# Autodesk Inventor assembly: 조립
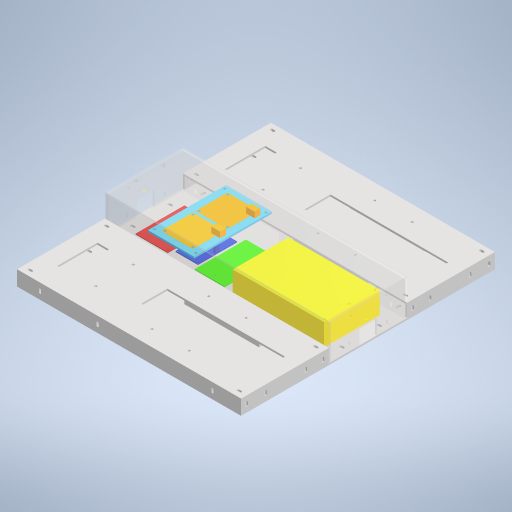
[picture p0: Inventor's stored thumbnail of the model, 512x512]
Saved by Autodesk Inventor 2024 (Build 280153000, 153)
## iProperties
Created: 2024-04-10
Part Number: 조립
Document SubType Name: Assembly
Designer: ckhye
Author: ckhye
## iProperties of the stored document 라즈베리파이.ipt
Created: 2024-06-01
Part Number: 라즈베리파이
Material: Generic
Document SubType Name: Modeling
Designer: ckhye
Density: 1 g/cm^3
Appearance: 기본값
Sending System: Autodesk Inventor 2025
Author: ckhye
## iProperties of the stored document 모터드라이버.ipt
Created: 2024-06-01
Part Number: 모터드라이버
Material: Generic
Document SubType Name: Modeling
Designer: ckhye
Density: 1 g/cm^3
Appearance: 기본값
Sending System: Autodesk Inventor 2025
Author: ckhye
## iProperties of the stored document 컨버터.ipt
Created: 2024-06-01
Part Number: 컨버터
Material: Generic
Document SubType Name: Modeling
Designer: ckhye
Density: 1 g/cm^3
Appearance: 기본값
Sending System: Autodesk Inventor 2025
Author: ckhye
## iProperties of the stored document SMPS.ipt
Created: 2024-06-01
Part Number: SMPS
Material: Generic
Document SubType Name: Modeling
Designer: ckhye
Density: 1 g/cm^3
Appearance: 기본값
Sending System: Autodesk Inventor 2025
Author: ckhye
## iProperties of the stored document 빵판.ipt
Created: 2024-06-01
Part Number: 빵판
Material: Generic
Document SubType Name: Modeling
Designer: ckhye
Density: 1 g/cm^3
Appearance: 기본값
Sending System: Autodesk Inventor 2025
Author: ckhye
## Documents named in this file (20)
- C:\Users\kkamin5\OneDrive - UOS\문서\Inventor\EBS project\모델링최종\조립.iam
- C:\Users\kkamin5\OneDrive - UOS\문서\Inventor\EBS project\모델링최종\발 받침대 받침_밑면.ipt
- C:\Users\kkamin5\OneDrive - UOS\문서\Inventor\EBS project\모델링최종\발 받침대 받침_위,아래.ipt
- C:\Users\kkamin5\OneDrive - UOS\문서\Inventor\EBS project\모델링최종\발 받침대 받침_좌,우.ipt
- C:\Users\kkamin5\OneDrive - UOS\문서\Inventor\EBS project\모델링최종\3D지지대.ipt
- C:\Users\kkamin5\OneDrive - UOS\문서\Inventor\EBS project\모델링최종\라즈베리파이보관_옆판.ipt
- C:\Users\kkamin5\OneDrive - UOS\문서\Inventor\EBS project\모델링최종\발받침대받침옆판.ipt
- C:\Users\kkamin5\OneDrive - UOS\문서\Inventor\EBS project\모델링최종\라즈베리파이보관_윗판.ipt
- C:\Users\kkamin5\OneDrive - UOS\문서\Inventor\EBS project\모델링최종\발 받침대 받침_윗면.ipt
- **C:\Users\kkamin5\OneDrive - UOS\문서\Inventor\EBS project\모델링최종\조립.iam*LocalDocs*xAaaaatbaAaaaaaaaAaaaqs4bRc*SMPS.ipt
- **C:\Users\kkamin5\OneDrive - UOS\문서\Inventor\EBS project\모델링최종\조립.iam*LocalDocs*xAaaaakbaAaaaaaaaAaaaqwuvSe*라즈베리파이.ipt
- **C:\Users\kkamin5\OneDrive - UOS\문서\Inventor\EBS project\모델링최종\조립.iam*LocalDocs*xAaaaqkbaAaaaaaaaAaaaamyz2g*빵판.ipt
- **C:\Users\kkamin5\OneDrive - UOS\문서\Inventor\EBS project\모델링최종\조립.iam*LocalDocs*xAaaaajbaAaaaaaaaAaaaag3xYb*모터드라이버.ipt
- **C:\Users\kkamin5\OneDrive - UOS\문서\Inventor\EBS project\모델링최종\조립.iam*LocalDocs*xAaaaqjbaAaaaaaaaAaaaqjrfGf*컨버터.ipt
- C:\Users\kkamin5\OneDrive - UOS\문서\Inventor\EBS project\모델링최종\라즈베리파이 보관소 2층 판.ipt
- C:\Users\kkamin5\OneDrive - UOS\문서\Inventor\EBS project\모델링최종\SMPS.ipt
- C:\Users\kkamin5\OneDrive - UOS\문서\Inventor\EBS project\모델링최종\라즈베리파이.ipt
- C:\Users\kkamin5\OneDrive - UOS\문서\Inventor\EBS project\모델링최종\빵판.ipt
- C:\Users\kkamin5\OneDrive - UOS\문서\Inventor\EBS project\모델링최종\모터드라이버.ipt
- C:\Users\kkamin5\OneDrive - UOS\문서\Inventor\EBS project\모델링최종\컨버터.ipt
## Components (27 placed, 14 different names)
1. 발 받침대 받침_밑면:1 — 메이트:1, 플러쉬:1, 메이트:2, 메이트:3, 플러쉬:3, 메이트:4, 플러쉬:5, 메이트:5, 플러쉬:6, 플러쉬:8, 메이트:7, 메이트:8, 플러쉬:10, 플러쉬:11, 플러쉬:12, 플러쉬:13, 메이트:13, 메이트:14, 메이트:15, 메이트:16, 메이트:17, 메이트:18, 메이트:35, 메이트:36, 메이트:38, 플러쉬:20, 플러쉬:22, 플러쉬:23, 메이트:67, 메이트:69, 메이트:76, 메이트:87, 메이트:92, 메이트:93, 메이트:94, 메이트:95, 메이트:96, 메이트:97, 메이트:98, 메이트:99, 메이트:100, 메이트:101, 메이트:102, 메이트:103
2. 발 받침대 받침_위,아래:1 — 메이트:3, 플러쉬:3, 메이트:10, 메이트:19
3. 발 받침대 받침_위,아래:2 — 메이트:4, 플러쉬:5, 메이트:9, 메이트:50
4. 발 받침대 받침_위,아래:3 — 메이트:5, 플러쉬:6, 메이트:12, 메이트:54, 플러쉬:30
5. 발 받침대 받침_위,아래:4 — 플러쉬:8, 메이트:27, 메이트:87, 메이트:88
6. 발 받침대 받침_좌,우:2 — 메이트:8, 플러쉬:12, 플러쉬:13, 메이트:12, 메이트:29, 플러쉬:29, 메이트:88
7. 발 받침대 받침_좌,우:4 — 메이트:7, 플러쉬:10, 플러쉬:11, 메이트:9, 메이트:10, 메이트:24, 메이트:53, 플러쉬:26, 플러쉬:27
8. 3D지지대:1 — 메이트:14, 메이트:60, 메이트:61
9. 3D지지대:2 — 메이트:16, 메이트:27, 메이트:29
10. 3D지지대:3 — 메이트:13, 메이트:62, 메이트:63
11. 3D지지대:4 — 메이트:17, 메이트:56, 메이트:57
12. 3D지지대:5 — 메이트:15, 메이트:58, 메이트:59
13. 3D지지대:6 — 메이트:18, 메이트:19, 메이트:24
14. 라즈베리파이보관_옆판:1 — 메이트:35, 플러쉬:22, 메이트:50, 플러쉬:25, 메이트:55, 메이트:84, 플러쉬:34, 플러쉬:35, 메이트:91
15. 라즈베리파이보관_옆판:2 — 메이트:36, 플러쉬:23, 메이트:52, 메이트:78, 메이트:83, 플러쉬:38
16. 발받침대받침옆판:1 — 메이트:38, 플러쉬:20, 메이트:55, 플러쉬:33
17. 라즈베리파이보관_윗판:1 — 메이트:52, 플러쉬:25, 메이트:85, 플러쉬:36
18. 발 받침대 받침_윗면:1 — 메이트:54, 플러쉬:29, 플러쉬:30, 메이트:60, 메이트:61, 메이트:62, 메이트:63
19. 발받침대받침옆판:2 — 메이트:83, 메이트:84, 플러쉬:34, 플러쉬:35, 메이트:85, 메이트:86, 플러쉬:36
20. SMPS:1 — 메이트:67, 메이트:78, 메이트:86
21. 라즈베리파이:1 — 메이트:69, 메이트:92, 메이트:93, 메이트:94, 메이트:95
22. 빵판:1 — 메이트:101, 메이트:102, 메이트:103
23. 모터드라이버:1 — 메이트:77, 플러쉬:32, 메이트:90
24. 컨버터:1 — 메이트:96, 메이트:97, 메이트:98, 메이트:99, 메이트:100
25. 라즈베리파이 보관소 2층 판:1 — 메이트:76, 메이트:77, 플러쉬:32, 플러쉬:33, 메이트:89, 플러쉬:37, 플러쉬:38
26. 모터드라이버:2 — 메이트:89, 플러쉬:37, 메이트:90, 메이트:91
27. 발 받침대 받침_윗면:2 — 메이트:53, 플러쉬:26, 플러쉬:27, 메이트:56, 메이트:57, 메이트:58, 메이트:59
## Relationships (86: Mate 62, Flush 24)
- 메이트:1 [Mate]: 발 받침대 받침_밑면:1
- 플러쉬:1 [Flush]: 발 받침대 받침_밑면:1
- 메이트:2 [Mate]: 발 받침대 받침_밑면:1
- 메이트:3 [Mate]: 발 받침대 받침_밑면:1 ↔ 발 받침대 받침_위,아래:1
- 플러쉬:3 [Flush]: 발 받침대 받침_밑면:1 ↔ 발 받침대 받침_위,아래:1
- 메이트:4 [Mate]: 발 받침대 받침_밑면:1 ↔ 발 받침대 받침_위,아래:2
- 플러쉬:5 [Flush]: 발 받침대 받침_밑면:1 ↔ 발 받침대 받침_위,아래:2
- 메이트:5 [Mate]: 발 받침대 받침_밑면:1 ↔ 발 받침대 받침_위,아래:3
- 플러쉬:6 [Flush]: 발 받침대 받침_밑면:1 ↔ 발 받침대 받침_위,아래:3
- 플러쉬:8 [Flush]: 발 받침대 받침_밑면:1 ↔ 발 받침대 받침_위,아래:4
- 메이트:7 [Mate]: 발 받침대 받침_밑면:1 ↔ 발 받침대 받침_좌,우:4
- 메이트:8 [Mate]: 발 받침대 받침_밑면:1 ↔ 발 받침대 받침_좌,우:2
- 플러쉬:10 [Flush]: 발 받침대 받침_밑면:1 ↔ 발 받침대 받침_좌,우:4
- 플러쉬:11 [Flush]: 발 받침대 받침_밑면:1 ↔ 발 받침대 받침_좌,우:4
- 플러쉬:12 [Flush]: 발 받침대 받침_밑면:1 ↔ 발 받침대 받침_좌,우:2
- 플러쉬:13 [Flush]: 발 받침대 받침_밑면:1 ↔ 발 받침대 받침_좌,우:2
- 메이트:9 [Mate]: 발 받침대 받침_위,아래:2 ↔ 발 받침대 받침_좌,우:4
- 메이트:10 [Mate]: 발 받침대 받침_위,아래:1 ↔ 발 받침대 받침_좌,우:4
- 메이트:12 [Mate]: 발 받침대 받침_위,아래:3 ↔ 발 받침대 받침_좌,우:2
- 메이트:13 [Mate]: 발 받침대 받침_밑면:1 ↔ 3D지지대:3
- 메이트:14 [Mate]: 발 받침대 받침_밑면:1 ↔ 3D지지대:1
- 메이트:15 [Mate]: 발 받침대 받침_밑면:1 ↔ 3D지지대:5
- 메이트:16 [Mate]: 발 받침대 받침_밑면:1 ↔ 3D지지대:2
- 메이트:17 [Mate]: 발 받침대 받침_밑면:1 ↔ 3D지지대:4
- 메이트:18 [Mate]: 발 받침대 받침_밑면:1 ↔ 3D지지대:6
- 메이트:19 [Mate] (81 mm): 발 받침대 받침_위,아래:1 ↔ 3D지지대:6
- 메이트:24 [Mate] (7.5 mm): 발 받침대 받침_좌,우:4 ↔ 3D지지대:6
- 메이트:27 [Mate] (81 mm): 발 받침대 받침_위,아래:4 ↔ 3D지지대:2
- 메이트:29 [Mate] (7.5 mm): 발 받침대 받침_좌,우:2 ↔ 3D지지대:2
- 메이트:35 [Mate]: 발 받침대 받침_밑면:1 ↔ 라즈베리파이보관_옆판:1
- 메이트:36 [Mate]: 발 받침대 받침_밑면:1 ↔ 라즈베리파이보관_옆판:2
- 메이트:38 [Mate]: 발 받침대 받침_밑면:1 ↔ 발받침대받침옆판:1
- 플러쉬:20 [Flush]: 발 받침대 받침_밑면:1 ↔ 발받침대받침옆판:1
- 플러쉬:22 [Flush]: 발 받침대 받침_밑면:1 ↔ 라즈베리파이보관_옆판:1
- 메이트:50 [Mate]: 발 받침대 받침_위,아래:2 ↔ 라즈베리파이보관_옆판:1
- 플러쉬:23 [Flush]: 발 받침대 받침_밑면:1 ↔ 라즈베리파이보관_옆판:2
- 메이트:52 [Mate]: 라즈베리파이보관_옆판:2 ↔ 라즈베리파이보관_윗판:1
- 플러쉬:25 [Flush]: 라즈베리파이보관_옆판:1 ↔ 라즈베리파이보관_윗판:1
- 메이트:53 [Mate]: 발 받침대 받침_좌,우:4 ↔ 발 받침대 받침_윗면:2
- 플러쉬:26 [Flush]: 발 받침대 받침_좌,우:4 ↔ 발 받침대 받침_윗면:2
- 플러쉬:27 [Flush]: 발 받침대 받침_좌,우:4 ↔ 발 받침대 받침_윗면:2
- 메이트:54 [Mate]: 발 받침대 받침_위,아래:3 ↔ 발 받침대 받침_윗면:1
- 플러쉬:29 [Flush]: 발 받침대 받침_좌,우:2 ↔ 발 받침대 받침_윗면:1
- 플러쉬:30 [Flush]: 발 받침대 받침_위,아래:3 ↔ 발 받침대 받침_윗면:1
- 메이트:55 [Mate]: 라즈베리파이보관_옆판:1 ↔ 발받침대받침옆판:1
- 메이트:56 [Mate]: 3D지지대:4 ↔ 발 받침대 받침_윗면:2
- 메이트:57 [Mate]: 3D지지대:4 ↔ 발 받침대 받침_윗면:2
- 메이트:58 [Mate]: 3D지지대:5 ↔ 발 받침대 받침_윗면:2
- 메이트:59 [Mate]: 3D지지대:5 ↔ 발 받침대 받침_윗면:2
- 메이트:60 [Mate]: 3D지지대:1 ↔ 발 받침대 받침_윗면:1
- 메이트:61 [Mate]: 3D지지대:1 ↔ 발 받침대 받침_윗면:1
- 메이트:62 [Mate]: 3D지지대:3 ↔ 발 받침대 받침_윗면:1
- 메이트:63 [Mate]: 3D지지대:3 ↔ 발 받침대 받침_윗면:1
- 메이트:67 [Mate]: 발 받침대 받침_밑면:1 ↔ SMPS:1
- 메이트:69 [Mate]: 발 받침대 받침_밑면:1 ↔ 라즈베리파이:1
- 메이트:76 [Mate] (40 mm): 발 받침대 받침_밑면:1 ↔ 라즈베리파이 보관소 2층 판:1
- 메이트:77 [Mate]: 모터드라이버:1 ↔ 라즈베리파이 보관소 2층 판:1
- 메이트:78 [Mate] (16.5 mm): 라즈베리파이보관_옆판:2 ↔ SMPS:1
- 플러쉬:32 [Flush] (12.5 mm): 모터드라이버:1 ↔ 라즈베리파이 보관소 2층 판:1
- 플러쉬:33 [Flush] (75 mm): 발받침대받침옆판:1 ↔ 라즈베리파이 보관소 2층 판:1
- 메이트:83 [Mate]: 라즈베리파이보관_옆판:2 ↔ 발받침대받침옆판:2
- 메이트:84 [Mate]: 라즈베리파이보관_옆판:1 ↔ 발받침대받침옆판:2
- 플러쉬:34 [Flush]: 라즈베리파이보관_옆판:1 ↔ 발받침대받침옆판:2
- 플러쉬:35 [Flush]: 라즈베리파이보관_옆판:1 ↔ 발받침대받침옆판:2
- 메이트:85 [Mate]: 라즈베리파이보관_윗판:1 ↔ 발받침대받침옆판:2
- 메이트:86 [Mate] (25 mm): 발받침대받침옆판:2 ↔ SMPS:1
- 플러쉬:36 [Flush]: 라즈베리파이보관_윗판:1 ↔ 발받침대받침옆판:2
- 메이트:87 [Mate]: 발 받침대 받침_밑면:1 ↔ 발 받침대 받침_위,아래:4
- 메이트:88 [Mate]: 발 받침대 받침_위,아래:4 ↔ 발 받침대 받침_좌,우:2
- 메이트:89 [Mate]: 라즈베리파이 보관소 2층 판:1 ↔ 모터드라이버:2
- 플러쉬:37 [Flush] (12.5 mm): 라즈베리파이 보관소 2층 판:1 ↔ 모터드라이버:2
- 메이트:90 [Mate] (5 mm): 모터드라이버:1 ↔ 모터드라이버:2
- 메이트:91 [Mate] (7.5 mm): 라즈베리파이보관_옆판:1 ↔ 모터드라이버:2
- 플러쉬:38 [Flush]: 라즈베리파이보관_옆판:2 ↔ 라즈베리파이 보관소 2층 판:1
- 메이트:92 [Mate]: 발 받침대 받침_밑면:1 ↔ 라즈베리파이:1
- 메이트:93 [Mate]: 발 받침대 받침_밑면:1 ↔ 라즈베리파이:1
- 메이트:94 [Mate]: 발 받침대 받침_밑면:1 ↔ 라즈베리파이:1
- 메이트:95 [Mate]: 발 받침대 받침_밑면:1 ↔ 라즈베리파이:1
- 메이트:96 [Mate]: 발 받침대 받침_밑면:1 ↔ 컨버터:1
- 메이트:97 [Mate]: 발 받침대 받침_밑면:1 ↔ 컨버터:1
- 메이트:98 [Mate]: 발 받침대 받침_밑면:1 ↔ 컨버터:1
- 메이트:99 [Mate]: 발 받침대 받침_밑면:1 ↔ 컨버터:1
- 메이트:100 [Mate]: 발 받침대 받침_밑면:1 ↔ 컨버터:1
- 메이트:101 [Mate]: 발 받침대 받침_밑면:1 ↔ 빵판:1
- 메이트:102 [Mate]: 발 받침대 받침_밑면:1 ↔ 빵판:1
- 메이트:103 [Mate]: 발 받침대 받침_밑면:1 ↔ 빵판:1
